# Autodesk Inventor assembly: Assembly1
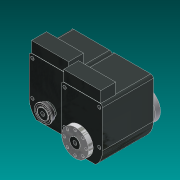
[picture p0: Inventor's stored thumbnail of the model, 180x180]
Saved by Autodesk Inventor 2015 (Build 190159000, 159)
## iProperties
Created: 2016-04-23
Part Number: Assembly1
Document SubType Name: Assembly
Designer: hiroaki
Author: hiroaki
## Documents named in this file (7)
- C:\Users\hiroaki\Documents\kenkyuu\二足\二足ver1.0\既製品\Assembly1.iam
- C:\Users\hiroaki\Documents\kenkyuu\二足\二足ver1.0\既製品\B3M10xx.ipt
- B3M11xx.ipt
- C:\Users\hiroaki\Documents\kenkyuu\二足\二足ver1.0\既製品\free_horn.ipt
- C:\Users\hiroaki\Documents\kenkyuu\二足\二足ver1.0\既製品\B3M11xx.ipt
- C:\Users\hiroaki\Documents\kenkyuu\二足\二足ver1.0\下半身\リンク\リンクスペーサ_1_1.ipt
- C:\Users\hiroaki\Documents\kenkyuu\二足\二足ver1.0\既製品\NSK_RB_MF128ZZ1\MF128ZZ1.iam
## Components (5 placed, 4 different names)
1. B3M11xx:1 — フラッシュ:1, メイト:1, フラッシュ:2, 挿入:5
2. B3M11xx:2 — フラッシュ:1, メイト:1, フラッシュ:2, 挿入:2, 挿入:3, 挿入:4
3. free_horn:2 — 挿入:2
4. リンクスペーサ_1_1:1 — 挿入:3, 挿入:4
5. MF128ZZ1:1 [sub-assembly] — 挿入:5
## Relationships (7: Insert 4, Flush 2, Mate 1)
- フラッシュ:1 [Flush]: B3M11xx:1 ↔ B3M11xx:2
- メイト:1 [Mate]: B3M11xx:1 ↔ B3M11xx:2
- フラッシュ:2 [Flush]: B3M11xx:1 ↔ B3M11xx:2
- 挿入:2 [Insert]: B3M11xx:2 ↔ free_horn:2
- 挿入:3 [Insert]: B3M11xx:2 ↔ リンクスペーサ_1_1:1
- 挿入:4 [Insert]: B3M11xx:2 ↔ リンクスペーサ_1_1:1
- 挿入:5 [Insert]: B3M11xx:1 ↔ MF128ZZ1:1
